# Autodesk Inventor assembly: Thigh-40x
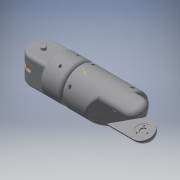
[picture p0: Inventor's stored thumbnail of the model, 180x180]
Saved by Autodesk Inventor 2018 (Build 220112000, 112)
## iProperties
Part Number: Thigh-40x
Material: Generisch
Document SubType Name: Assembly
Designer: Jochen Alt
Mass: 186.402 g
Surface Area: 1060.57 cm^2
Volume: 140.56 cm^3
Density: 1.32614 g/cm^3
Author: Jochen Alt
## Documents named in this file (8)
- D:\Projects\Manfred\design\cad\Inventor\Thigh-40x.iam
- D:\Projects\Manfred\design\cad\Inventor\Thigh Bushing.ipt
- D:\Projects\Manfred\design\cad\Inventor\Oberschenkel\Konstruktions-Assistent\Kegelräder1.iam
- D:\Projects\Manfred\design\cad\Inventor\Herkulex DRS-010x\W 61707-2RS1.ipt
- D:\Projects\Manfred\design\cad\Inventor\Rillenkugellager 11x7x3 inafag smr117.ipt
- D:\Projects\Manfred\design\cad\Inventor\Thigh-40x.ipt
- D:\Projects\Manfred\design\cad\Inventor\Herkulex DRS-040x.ipt
- D:\Projects\Manfred\design\cad\Inventor\Knee-40x.ipt
## Components (7 placed, 7 different names)
1. Thigh Bushing:1 — Passend:30, Passend:31, Passend:47, Passend:56
2. Kegelräder:2 [sub-assembly] — Passend:56, Passend:57, Passend:58, Passend:61, Winkel:1, Passend:62
3. W 61707-2RS1:1 — Passend:30, Passend:31, Passend:44, Passend:54
4. Rillenkugellager 11x7x3 inafag smr117:2 — Passend:57, Passend:58
5. Thigh-40x:1 — Passend:44, Passend:54, Winkel:1, Passend:62, Winkel:2, Fluchtend:1, Passend:64, Winkel:3
6. Herkulex DRS-040x:1 — Winkel:2, Fluchtend:1, Passend:64
7. Knee-40x:1 — Passend:47, Passend:61
## Relationships (15: Mate 11, Angle 3, Flush 1)
- Passend:30 [Mate]: Thigh Bushing:1 ↔ W 61707-2RS1:1
- Passend:31 [Mate]: Thigh Bushing:1 ↔ W 61707-2RS1:1
- Passend:44 [Mate]: W 61707-2RS1:1 ↔ Thigh-40x:1
- Passend:47 [Mate]: Thigh Bushing:1 ↔ Knee-40x:1
- Passend:54 [Mate]: W 61707-2RS1:1 ↔ Thigh-40x:1
- Passend:56 [Mate]: Thigh Bushing:1 ↔ Kegelräder:2
- Passend:57 [Mate]: Kegelräder:2 ↔ Rillenkugellager 11x7x3 inafag smr117:2
- Passend:58 [Mate]: Kegelräder:2 ↔ Rillenkugellager 11x7x3 inafag smr117:2
- Passend:61 [Mate]: Kegelräder:2 ↔ Knee-40x:1
- Winkel:1 [Angle] (180 deg): Kegelräder:2 ↔ Thigh-40x:1
- Passend:62 [Mate]: Kegelräder:2 ↔ Thigh-40x:1
- Winkel:2 [Angle] (180 deg): Thigh-40x:1 ↔ Herkulex DRS-040x:1
- Fluchtend:1 [Flush] (0.2 mm): Thigh-40x:1 ↔ Herkulex DRS-040x:1
- Passend:64 [Mate]: Thigh-40x:1 ↔ Herkulex DRS-040x:1
- Winkel:3 [Angle] (0 deg): Thigh-40x:1
